# Autodesk Inventor assembly: Full_Design
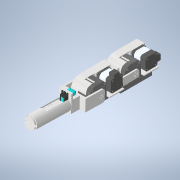
[picture p0: Inventor's stored thumbnail of the model, 180x180]
Saved by Autodesk Inventor 2022 (Build 260153000, 153)
## iProperties
Created: 2022-02-25
Part Number: Full_Design
Document SubType Name: Assembly
Designer: Mlees
Author: Mlees
## Documents named in this file (27)
- C:\Users\Mlees\Desktop\504Engineering\Stepper-Servo_Based_Robotic_Arm\Designs\Version_7\Full_Design.iam
- C:\Users\Mlees\Desktop\504Engineering\Stepper-Servo_Based_Robotic_Arm\Designs\Version_7\Created_Parts\24_Teeth_Sun_Gear.ipt
- C:\Users\Mlees\Desktop\504Engineering\Stepper-Servo_Based_Robotic_Arm\Designs\Version_7\Created_Parts\36_Teeth_Planet_Gear.ipt
- C:\Users\Mlees\Desktop\504Engineering\Stepper-Servo_Based_Robotic_Arm\Designs\Version_7\Created_Parts\Joint1.ipt
- C:\Users\Mlees\Desktop\504Engineering\Stepper-Servo_Based_Robotic_Arm\Designs\Version_7\Created_Parts\Plamet_Carrier.ipt
- C:\Users\Mlees\Desktop\504Engineering\Stepper-Servo_Based_Robotic_Arm\Designs\Version_7\Created_Parts\Planet_Carrier_Modifed_with_sun_gear.ipt
- C:\Users\Mlees\Desktop\504Engineering\Stepper-Servo_Based_Robotic_Arm\Designs\Version_7\Created_Parts\Gear_Cover_modified.ipt
- C:\Users\Mlees\Desktop\504Engineering\Stepper-Servo_Based_Robotic_Arm\Designs\Version_7\Created_Parts\Combined_Gear_Box_Modified_2.ipt
- C:\Users\Mlees\Desktop\504Engineering\Stepper-Servo_Based_Robotic_Arm\Designs\Version_7\Downloaded_Parts\GT2 20T Drive Pulley.ipt
- C:\Users\Mlees\Desktop\504Engineering\Stepper-Servo_Based_Robotic_Arm\Designs\Version_7\Downloaded_Parts\GT2 60T Drive Pulley.ipt
- C:\Users\Mlees\Desktop\504Engineering\Stepper-Servo_Based_Robotic_Arm\Designs\Version_7\Downloaded_Parts\9403T15_Tight-Tolerance High-Strength 7075 Aluminum Rod.ipt
- C:\Users\Mlees\Desktop\504Engineering\Stepper-Servo_Based_Robotic_Arm\Designs\Version_7\Downloaded_Parts\91290A059_Black-Oxide Alloy Steel Socket Head Screw_M3_30mm.ipt
- C:\Users\Mlees\Desktop\504Engineering\Stepper-Servo_Based_Robotic_Arm\Designs\Version_7\Downloaded_Parts\124125202-9-stp-mtr-17040w\stp-mtr-17040w.ipt
- C:\Users\Mlees\Desktop\504Engineering\Stepper-Servo_Based_Robotic_Arm\Designs\Version_7\Downloaded_Parts\nema17-speed-reducer-1.snapshot.9\M3 Insert 5D x 6L.step.ipt
- C:\Users\Mlees\Desktop\504Engineering\Stepper-Servo_Based_Robotic_Arm\Designs\Version_7\Created_Parts\Combined_Gear_Box_Modified_3.ipt
- C:\Users\Mlees\Desktop\504Engineering\Stepper-Servo_Based_Robotic_Arm\Designs\Version_7\Downloaded_Parts\uploads_files_140274_ServoSW-1211SG.ipt
- C:\Users\Mlees\Desktop\504Engineering\Stepper-Servo_Based_Robotic_Arm\Designs\Version_7\Created_Parts\Metal_AttachmentBracket.ipt
- C:\Users\Mlees\Desktop\504Engineering\Stepper-Servo_Based_Robotic_Arm\Designs\Version_7\Created_Parts\Tilt_Bracket_Output_2.ipt
- C:\Users\Mlees\Desktop\504Engineering\Stepper-Servo_Based_Robotic_Arm\Designs\Version_7\Created_Parts\Belt_Bearing_Holder.ipt
- C:\Users\Mlees\Desktop\504Engineering\Stepper-Servo_Based_Robotic_Arm\Designs\Version_7\Created_Parts\Belt_Bearing_Holder_p2.ipt
- C:\Users\Mlees\Desktop\504Engineering\Stepper-Servo_Based_Robotic_Arm\Designs\Version_7\Created_Parts\Belt_Tension_Bearing.ipt
- C:\Users\Mlees\Desktop\504Engineering\Stepper-Servo_Based_Robotic_Arm\Designs\Version_7\Created_Parts\Twist_Attachment_To_Servo_Horn.ipt
- C:\Users\Mlees\Desktop\504Engineering\Stepper-Servo_Based_Robotic_Arm\Designs\Version_7\Created_Parts\Twist_Servo_Horn.ipt
- C:\Users\Mlees\Desktop\504Engineering\Stepper-Servo_Based_Robotic_Arm\Designs\Version_7\Created_Parts\Twist_Rod.ipt
- C:\Users\Mlees\Desktop\504Engineering\Stepper-Servo_Based_Robotic_Arm\Designs\Version_7\Created_Parts\Tilt_Bracket_Output_2_Lid.ipt
- C:\Users\Mlees\Desktop\504Engineering\Stepper-Servo_Based_Robotic_Arm\Designs\Version_7\Created_Parts\Claw_Attachment.ipt
- C:\Users\Mlees\Desktop\504Engineering\Stepper-Servo_Based_Robotic_Arm\Designs\Version_7\Created_Parts\Bearing_Holder.ipt
## Components (67 placed, 26 different names)
1. 24_Teeth_Sun_Gear:1 — Rigid:20, Rotational:33
2. 36_Teeth_Planet_Gear:1 — Rotational:18
3. 36_Teeth_Planet_Gear:2 — Rotational:17
4. 36_Teeth_Planet_Gear:3 — Rotational:16
5. 36_Teeth_Planet_Gear:4 — Rotational:15
6. 36_Teeth_Planet_Gear:5 — Rotational:14
7. 36_Teeth_Planet_Gear:6 — Rotational:13
8. Joint1:1 — Rigid:12, Rigid:13, Rigid:18, Rotational:26, Rigid:23, Rotational:35, Rotational:38, Rotational:43
9. Plamet_Carrier:1 — Rotational:16, Rotational:17, Rotational:18, Rotational:20
10. Planet_Carrier_Modifed_with_sun_gear:1 — Rotational:13, Rotational:14, Rotational:15, Rotational:19, Rotational:20
11. Gear_Cover_modified:1 — Rotational:21
12. Combined_Gear_Box_Modified_2:1 — Rigid:4, Rigid:5, Rigid:6, Rigid:7, Rigid:8, Rotational:3, Rotational:21, Rotational:22, Rotational:23
13. GT2 20T Drive Pulley:1 — Rotational:1
14. GT2 60T Drive Pulley:1 — Rigid:10, Rotational:4
15. 9403T15_Tight-Tolerance High-Strength 7075 Aluminum Rod:1 — Rigid:11, Rigid:19
16. 91290A059_Black-Oxide Alloy Steel Socket Head Screw_M3_30mm:1 — Rotational:23
17. 91290A059_Black-Oxide Alloy Steel Socket Head Screw_M3_30mm:2 — Rotational:25
18. stp-mtr-17040w:1 — Rotational:2, Rigid:24
19. stp-mtr-17040w:2 — Rotational:1, Rigid:22
20. M3 Insert 5D x 6L.step:1 — Rigid:2
21. M3 Insert 5D x 6L.step:2 — Rigid:3
22. M3 Insert 5D x 6L.step:3 — Rigid:4
23. M3 Insert 5D x 6L.step:4 — Rigid:6
24. M3 Insert 5D x 6L.step:5 — Rigid:5
25. M3 Insert 5D x 6L.step:6 — Rigid:7
26. M3 Insert 5D x 6L.step:7 — Rigid:12
27. M3 Insert 5D x 6L.step:8 — Rigid:13
28. M3 Insert 5D x 6L.step:9 — Rigid:14
29. M3 Insert 5D x 6L.step:10 — Rigid:15
30. M3 Insert 5D x 6L.step:11 — Rigid:16
31. M3 Insert 5D x 6L.step:12 — Rigid:17
32. Combined_Gear_Box_Modified_2:2 — Rigid:14, Rigid:15, Rigid:16, Rigid:17, Rigid:18, Rotational:4, Rotational:24, Rotational:25, Rigid:21
33. Combined_Gear_Box_Modified_3:1 — Rigid:2, Rigid:3, Rigid:8, Rotational:26, Rigid:25, Rigid:34
34. GT2 20T Drive Pulley:2 — Rotational:2
35. GT2 60T Drive Pulley:2 — Rigid:11, Rotational:3
36. 9403T15_Tight-Tolerance High-Strength 7075 Aluminum Rod:2 — Rigid:10, Rigid:20
37. 24_Teeth_Sun_Gear:2 — Rigid:19, Rotational:19
38. 91290A059_Black-Oxide Alloy Steel Socket Head Screw_M3_30mm:3 — Rotational:22
39. 91290A059_Black-Oxide Alloy Steel Socket Head Screw_M3_30mm:4 — Rotational:24
40. 36_Teeth_Planet_Gear:7 — Rotational:32
41. Plamet_Carrier:2 — Rotational:30, Rotational:31, Rotational:32, Rotational:34
42. Planet_Carrier_Modifed_with_sun_gear:2 — Rotational:27, Rotational:28, Rotational:29, Rotational:33, Rotational:34
43. 36_Teeth_Planet_Gear:8 — Rotational:31
44. 36_Teeth_Planet_Gear:9 — Rotational:29
45. 36_Teeth_Planet_Gear:10 — Rotational:30
46. 36_Teeth_Planet_Gear:11 — Rotational:27
47. 36_Teeth_Planet_Gear:12 — Rotational:28
48. Gear_Cover_modified:2 — Rigid:21
49. Metal_AttachmentBracket:1 — Rigid:22, Rigid:23
50. Metal_AttachmentBracket:2 — Rigid:24, Rigid:25
51. Tilt_Bracket_Output_2:1 — Rotational:35, Rigid:27, Rigid:33
52. Belt_Bearing_Holder:1 — Rotational:36, Rigid:26, Rotational:38
53. Belt_Bearing_Holder_p2:1 — Rigid:26
54. Belt_Tension_Bearing:1 — Rotational:36, Rotational:37
55. Belt_Tension_Bearing:3 — Rotational:37
56. uploads_files_140274_ServoSW-1211SG:1 — Rigid:27, Rigid:29
57. Twist_Attachment_To_Servo_Horn:1 — Rigid:28, Rigid:30
58. Twist_Servo_Horn:1 — Rigid:28, Rigid:29
59. Twist_Rod:1 — Rigid:30, Rigid:32
60. Tilt_Bracket_Output_2_Lid:1 — Rigid:33
61. Claw_Attachment:1 — Rigid:32
62. Bearing_Holder:1 — Rotational:41, Rotational:42, Rotational:43
63. Bearing_Holder:2 — Rotational:39, Rigid:34
64. Belt_Tension_Bearing:4 — Rotational:39, Rotational:40
65. Belt_Tension_Bearing:5 — Rotational:40
66. Belt_Tension_Bearing:6 — Rotational:42
67. Belt_Tension_Bearing:7 — Rotational:41
## Relationships (66: RevoluteJoint 35, WeldJoint 31)
- Rotational:1 [RevoluteJoint]: GT2 20T Drive Pulley:1 ↔ stp-mtr-17040w:2
- Rotational:2 [RevoluteJoint]: stp-mtr-17040w:1 ↔ GT2 20T Drive Pulley:2
- Rigid:2 [WeldJoint]: M3 Insert 5D x 6L.step:1 ↔ Combined_Gear_Box_Modified_3:1
- Rigid:3 [WeldJoint]: M3 Insert 5D x 6L.step:2 ↔ Combined_Gear_Box_Modified_3:1
- Rigid:4 [WeldJoint]: Combined_Gear_Box_Modified_2:1 ↔ M3 Insert 5D x 6L.step:3
- Rigid:5 [WeldJoint]: Combined_Gear_Box_Modified_2:1 ↔ M3 Insert 5D x 6L.step:5
- Rigid:6 [WeldJoint]: Combined_Gear_Box_Modified_2:1 ↔ M3 Insert 5D x 6L.step:4
- Rigid:7 [WeldJoint]: Combined_Gear_Box_Modified_2:1 ↔ M3 Insert 5D x 6L.step:6
- Rigid:8 [WeldJoint]: Combined_Gear_Box_Modified_2:1 ↔ Combined_Gear_Box_Modified_3:1
- Rigid:10 [WeldJoint]: GT2 60T Drive Pulley:1 ↔ 9403T15_Tight-Tolerance High-Strength 7075 Aluminum Rod:2
- Rigid:11 [WeldJoint]: 9403T15_Tight-Tolerance High-Strength 7075 Aluminum Rod:1 ↔ GT2 60T Drive Pulley:2
- Rigid:12 [WeldJoint]: Joint1:1 ↔ M3 Insert 5D x 6L.step:7
- Rigid:13 [WeldJoint]: Joint1:1 ↔ M3 Insert 5D x 6L.step:8
- Rigid:14 [WeldJoint]: M3 Insert 5D x 6L.step:9 ↔ Combined_Gear_Box_Modified_2:2
- Rigid:15 [WeldJoint]: M3 Insert 5D x 6L.step:10 ↔ Combined_Gear_Box_Modified_2:2
- Rigid:16 [WeldJoint]: M3 Insert 5D x 6L.step:11 ↔ Combined_Gear_Box_Modified_2:2
- Rigid:17 [WeldJoint]: M3 Insert 5D x 6L.step:12 ↔ Combined_Gear_Box_Modified_2:2
- Rigid:18 [WeldJoint]: Joint1:1 ↔ Combined_Gear_Box_Modified_2:2
- Rigid:19 [WeldJoint]: 9403T15_Tight-Tolerance High-Strength 7075 Aluminum Rod:1 ↔ 24_Teeth_Sun_Gear:2
- Rigid:20 [WeldJoint]: 24_Teeth_Sun_Gear:1 ↔ 9403T15_Tight-Tolerance High-Strength 7075 Aluminum Rod:2
- Rotational:3 [RevoluteJoint]: Combined_Gear_Box_Modified_2:1 ↔ GT2 60T Drive Pulley:2
- Rotational:4 [RevoluteJoint]: GT2 60T Drive Pulley:1 ↔ Combined_Gear_Box_Modified_2:2
- Rotational:13 [RevoluteJoint]: 36_Teeth_Planet_Gear:6 ↔ Planet_Carrier_Modifed_with_sun_gear:1
- Rotational:14 [RevoluteJoint]: 36_Teeth_Planet_Gear:5 ↔ Planet_Carrier_Modifed_with_sun_gear:1
- Rotational:15 [RevoluteJoint]: 36_Teeth_Planet_Gear:4 ↔ Planet_Carrier_Modifed_with_sun_gear:1
- Rotational:16 [RevoluteJoint]: 36_Teeth_Planet_Gear:3 ↔ Plamet_Carrier:1
- Rotational:17 [RevoluteJoint]: 36_Teeth_Planet_Gear:2 ↔ Plamet_Carrier:1
- Rotational:18 [RevoluteJoint]: 36_Teeth_Planet_Gear:1 ↔ Plamet_Carrier:1
- Rotational:19 [RevoluteJoint]: Planet_Carrier_Modifed_with_sun_gear:1 ↔ 24_Teeth_Sun_Gear:2
- Rotational:20 [RevoluteJoint]: Plamet_Carrier:1 ↔ Planet_Carrier_Modifed_with_sun_gear:1
- Rotational:21 [RevoluteJoint]: Gear_Cover_modified:1 ↔ Combined_Gear_Box_Modified_2:1
- Rotational:22 [RevoluteJoint]: Combined_Gear_Box_Modified_2:1 ↔ 91290A059_Black-Oxide Alloy Steel Socket Head Screw_M3_30mm:3
- Rotational:23 [RevoluteJoint]: Combined_Gear_Box_Modified_2:1 ↔ 91290A059_Black-Oxide Alloy Steel Socket Head Screw_M3_30mm:1
- Rotational:24 [RevoluteJoint]: Combined_Gear_Box_Modified_2:2 ↔ 91290A059_Black-Oxide Alloy Steel Socket Head Screw_M3_30mm:4
- Rotational:25 [RevoluteJoint]: 91290A059_Black-Oxide Alloy Steel Socket Head Screw_M3_30mm:2 ↔ Combined_Gear_Box_Modified_2:2
- Rotational:26 [RevoluteJoint]: Joint1:1 ↔ Combined_Gear_Box_Modified_3:1
- Rotational:27 [RevoluteJoint]: Planet_Carrier_Modifed_with_sun_gear:2 ↔ 36_Teeth_Planet_Gear:11
- Rotational:28 [RevoluteJoint]: Planet_Carrier_Modifed_with_sun_gear:2 ↔ 36_Teeth_Planet_Gear:12
- Rotational:29 [RevoluteJoint]: Planet_Carrier_Modifed_with_sun_gear:2 ↔ 36_Teeth_Planet_Gear:9
- Rotational:30 [RevoluteJoint]: Plamet_Carrier:2 ↔ 36_Teeth_Planet_Gear:10
- Rotational:31 [RevoluteJoint]: Plamet_Carrier:2 ↔ 36_Teeth_Planet_Gear:8
- Rotational:32 [RevoluteJoint]: 36_Teeth_Planet_Gear:7 ↔ Plamet_Carrier:2
- Rotational:33 [RevoluteJoint]: 24_Teeth_Sun_Gear:1 ↔ Planet_Carrier_Modifed_with_sun_gear:2
- Rotational:34 [RevoluteJoint]: Plamet_Carrier:2 ↔ Planet_Carrier_Modifed_with_sun_gear:2
- Rigid:21 [WeldJoint]: Combined_Gear_Box_Modified_2:2 ↔ Gear_Cover_modified:2
- Rigid:22 [WeldJoint]: stp-mtr-17040w:2 ↔ Metal_AttachmentBracket:1
- Rigid:23 [WeldJoint]: Joint1:1 ↔ Metal_AttachmentBracket:1
- Rigid:24 [WeldJoint]: stp-mtr-17040w:1 ↔ Metal_AttachmentBracket:2
- Rigid:25 [WeldJoint]: Combined_Gear_Box_Modified_3:1 ↔ Metal_AttachmentBracket:2
- Rotational:35 [RevoluteJoint]: Joint1:1 ↔ Tilt_Bracket_Output_2:1
- Rotational:36 [RevoluteJoint]: Belt_Bearing_Holder:1 ↔ Belt_Tension_Bearing:1
- Rotational:37 [RevoluteJoint]: Belt_Tension_Bearing:1 ↔ Belt_Tension_Bearing:3
- Rigid:26 [WeldJoint]: Belt_Bearing_Holder:1 ↔ Belt_Bearing_Holder_p2:1
- Rotational:38 [RevoluteJoint]: Joint1:1 ↔ Belt_Bearing_Holder:1
- Rigid:27 [WeldJoint]: Tilt_Bracket_Output_2:1 ↔ uploads_files_140274_ServoSW-1211SG:1
- Rigid:28 [WeldJoint]: Twist_Attachment_To_Servo_Horn:1 ↔ Twist_Servo_Horn:1
- Rigid:29 [WeldJoint]: uploads_files_140274_ServoSW-1211SG:1 ↔ Twist_Servo_Horn:1
- Rigid:30 [WeldJoint]: Twist_Attachment_To_Servo_Horn:1 ↔ Twist_Rod:1
- Rigid:32 [WeldJoint]: Twist_Rod:1 ↔ Claw_Attachment:1
- Rigid:33 [WeldJoint]: Tilt_Bracket_Output_2:1 ↔ Tilt_Bracket_Output_2_Lid:1
- Rotational:39 [RevoluteJoint]: Bearing_Holder:2 ↔ Belt_Tension_Bearing:4
- Rotational:40 [RevoluteJoint]: Belt_Tension_Bearing:4 ↔ Belt_Tension_Bearing:5
- Rotational:41 [RevoluteJoint]: Bearing_Holder:1 ↔ Belt_Tension_Bearing:7
- Rotational:42 [RevoluteJoint]: Bearing_Holder:1 ↔ Belt_Tension_Bearing:6
- Rigid:34 [WeldJoint]: Combined_Gear_Box_Modified_3:1 ↔ Bearing_Holder:2
- Rotational:43 [RevoluteJoint]: Joint1:1 ↔ Bearing_Holder:1
